# Autodesk Inventor assembly: Main
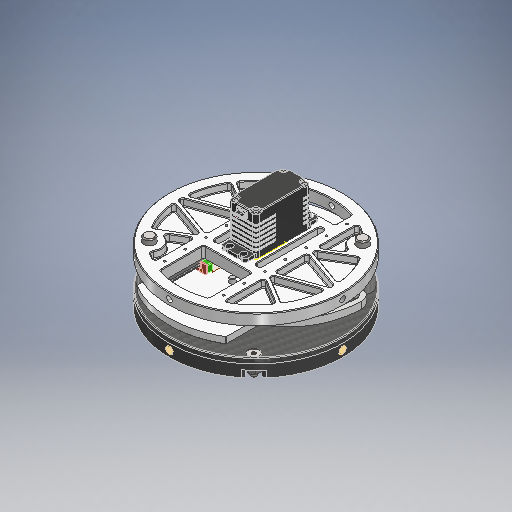
[picture p0: Inventor's stored thumbnail of the model, 512x512]
Saved by Autodesk Inventor 2027 (Build 310192060, 192F)
## iProperties
Created: 2026-06-20
Part Number: Main
Description: STEP AP242 Edition 2
Document SubType Name: Assembly
Designer: opore
Sending System: ONSHAPE BY PTC INC, 1.216
Preprocessor: ST-DEVELOPER v20
Title: Main
## Documents named in this file (20)
- C:\Users\opore\OneDrive\Desktop\Reducted-Airbrake\Optimized Airbrake\Main.iam
- C:\Users\opore\OneDrive\Desktop\Reducted-Airbrake\Optimized Airbrake\CAM.ipt
- C:\Users\opore\OneDrive\Desktop\Reducted-Airbrake\Optimized Airbrake\MANIFOLD_SOLID_BREP_40_1.ipt
- C:\Users\opore\OneDrive\Desktop\Reducted-Airbrake\Optimized Airbrake\Radial Thread insertup.ipt
- C:\Users\opore\OneDrive\Desktop\Reducted-Airbrake\Optimized Airbrake\JX BLS-HV7146MG.ipt
- C:\Users\opore\OneDrive\Desktop\Reducted-Airbrake\Optimized Airbrake\Spacer.ipt
- C:\Users\opore\OneDrive\Desktop\Reducted-Airbrake\Optimized Airbrake\1922-0025-0036 assembly.iam
- C:\Users\opore\OneDrive\Desktop\Reducted-Airbrake\Optimized Airbrake\MANIFOLD_SOLID_BREP_40_1_MIR3.ipt
- C:\Users\opore\OneDrive\Desktop\Reducted-Airbrake\Optimized Airbrake\Leafers.iam
- C:\Users\opore\OneDrive\Desktop\Reducted-Airbrake\Optimized Airbrake\1611-0514-4008.ipt
- C:\Users\opore\OneDrive\Desktop\Reducted-Airbrake\Optimized Airbrake\Leafers_MIR.iam
- C:\Users\opore\OneDrive\Desktop\Reducted-Airbrake\Optimized Airbrake\MiddleLand.ipt
- C:\Users\opore\OneDrive\Desktop\Reducted-Airbrake\Optimized Airbrake\3DprintRadial.ipt
- C:\Users\opore\OneDrive\Desktop\Reducted-Airbrake\Optimized Airbrake\M4x6mm_threaded_brass_insert.ipt
- C:\Users\opore\OneDrive\Documents\Inventor\Content Center Files\R2027\en-US\BS 4168(8)\BS 4168 - M3 x 25(7).ipt
- C:\Users\opore\OneDrive\Documents\Inventor\Content Center Files\R2027\en-US\ANSI B18.3.4M(2)\ANSI B18.3.4M - M8 x 1.25 x 45(1).ipt
- C:\Users\opore\OneDrive\Documents\Inventor\Content Center Files\R2027\en-US\ASME ANSI B18.3.5M(2)\ASME_ANSI B18.3.5M - M4x14(2).ipt
- C:\Users\opore\OneDrive\Documents\Inventor\Content Center Files\R2027\en-US\AS 1112 (2)\AS 1112 - M4  Type 5.ipt
- C:\Users\opore\OneDrive\Desktop\Reducted-Airbrake\Optimized Airbrake\Locking.iam
- C:\Users\opore\OneDrive\Desktop\Reducted-Airbrake\Optimized Airbrake\Spacers.ipt
## Components (26 placed, 19 different names)
1. Radial Thread insertup — Rigid:7, Rigid:10, Rigid:11, Flush:4, Flush:5
2. JX BLS-HV7146MG — Rotational:4, Rigid:7
3. Spacer:1
4. CAM:3 — Transitional:1, Transitional:2
5. 1922-0025-0036 assembly:2 [sub-assembly] — Rotational:4, Rigid:12, Rigid:14
6. MANIFOLD_SOLID_BREP_40_1:3 — Rigid:10, Slider:1, Slider:2
7. MANIFOLD_SOLID_BREP_40_1_MIR3:1 — Rigid:11
8. Leafers:1 [sub-assembly] — Slider:1, Transitional:2
9. 1611-0514-4008:1 — Rigid:12
10. Leafers_MIR:1 [sub-assembly] — Slider:2, Transitional:1
11. MiddleLand:1 — Rotational:6, Rigid:19, Flush:6, Flush:7, Rigid:20
12. 3DprintRadial:2 — Rotational:6, Flush:4, Flush:5, Rigid:13, Rigid:15, Rigid:16, Rigid:17, Rigid:18
13. BS 4168 : Part 8 Hexagon socket countersunk and button head screws - Metric series - Metric M3 x 25:1 — Rigid:14
14. Forged Hexagon Socket Button Head Cap Screw - Metric M8 x 1.25 x 45:1 — Rigid:15
15. Forged Hexagon Socket Button Head Cap Screw - Metric M8 x 1.25 x 45:2 — Rigid:16
16. Broached Hexagon Socket Flat Countersunk Head Cap Screws - Metric M4x14:1 — Rigid:19
17. Broached Hexagon Socket Flat Countersunk Head Cap Screws - Metric M4x14:2
18. AS 1112 (2) - Metric M4  Type 5:1 — Rigid:17
19. AS 1112 (2) - Metric M4  Type 5:2 — Rigid:18
20. Locking:1 [sub-assembly]
21. Spacers:1 — Flush:6, Flush:7
22. Spacers:2 — Rigid:20
23. M4x6mm_threaded_brass_insert:1 — Rigid:13
24. M4x6mm_threaded_brass_insert:2
25. M4x6mm_threaded_brass_insert:3
26. M4x6mm_threaded_brass_insert:4
## Component patterns: (4 elements, first: M4x6mm_threaded_brass_insert:1)
## Relationships (24: WeldJoint 14, Flush 4, RevoluteJoint 2, TranslationJoint 2, Transitional 2)
- Rotational:4 [RevoluteJoint]: JX BLS-HV7146MG ↔ 1922-0025-0036 assembly:2
- Rigid:7 [WeldJoint]: Radial Thread insertup ↔ JX BLS-HV7146MG
- [WeldJoint]: 1922-0025-0036 assembly:2 ↔ Locking:1
- [WeldJoint]: CAM:3 ↔ Locking:1
- Rigid:10 [WeldJoint]: Radial Thread insertup ↔ MANIFOLD_SOLID_BREP_40_1:3
- Rigid:11 [WeldJoint]: Radial Thread insertup ↔ MANIFOLD_SOLID_BREP_40_1_MIR3:1
- Slider:1 [TranslationJoint]: MANIFOLD_SOLID_BREP_40_1:3 ↔ Leafers:1
- Slider:2 [TranslationJoint]: MANIFOLD_SOLID_BREP_40_1:3 ↔ Leafers_MIR:1
- Transitional:1: CAM:3 ↔ Leafers_MIR:1
- Transitional:2: CAM:3 ↔ Leafers:1
- Rigid:12 [WeldJoint]: 1922-0025-0036 assembly:2 ↔ 1611-0514-4008:1
- Rotational:6 [RevoluteJoint]: MiddleLand:1 ↔ 3DprintRadial:2
- Flush:4: Radial Thread insertup ↔ 3DprintRadial:2
- Flush:5: Radial Thread insertup ↔ 3DprintRadial:2
- Rigid:13 [WeldJoint]: 3DprintRadial:2 ↔ M4x6mm_threaded_brass_insert:1
- Rigid:14 [WeldJoint]: 1922-0025-0036 assembly:2 ↔ BS 4168 : Part 8 Hexagon socket countersunk and button head screws - Metric series - Metric M3 x 25:1
- Rigid:15 [WeldJoint]: 3DprintRadial:2 ↔ Forged Hexagon Socket Button Head Cap Screw - Metric M8 x 1.25 x 45:1
- Rigid:16 [WeldJoint]: 3DprintRadial:2 ↔ Forged Hexagon Socket Button Head Cap Screw - Metric M8 x 1.25 x 45:2
- Rigid:17 [WeldJoint]: 3DprintRadial:2 ↔ AS 1112 (2) - Metric M4  Type 5:1
- Rigid:18 [WeldJoint]: 3DprintRadial:2 ↔ AS 1112 (2) - Metric M4  Type 5:2
- Rigid:19 [WeldJoint]: MiddleLand:1 ↔ Broached Hexagon Socket Flat Countersunk Head Cap Screws - Metric M4x14:1
- Flush:6: MiddleLand:1 ↔ Spacers:1
- Flush:7: MiddleLand:1 ↔ Spacers:1
- Rigid:20 [WeldJoint]: MiddleLand:1 ↔ Spacers:2
## Named parameters: Finish1_Area = 54.1838, Finish2_Area = 56.1125, Finish3_Area = 209.945
note: some values were not read from the file. Shown as the stored number, unit unknown: "Finish1_Area", "Finish2_Area", "Finish3_Area".
